# Autodesk Inventor assembly: inner
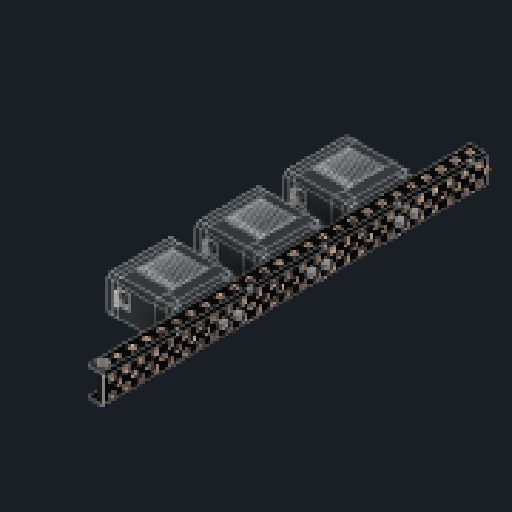
[picture p0: Inventor's stored thumbnail of the model, 512x512]
Saved by Autodesk Inventor 2024 (Build 280153000, 153)
## iProperties
Created: 2024-03-23
Part Number: inner
Document SubType Name: Assembly
Designer: Averey Ku
Author: Averey Ku
## Documents named in this file (8)
- D:\vex_robotics\hardware\cad\infection\chassis\drivebay\inner.iam
- D:\vex_robotics\hardware\cad\VEX-CAD-Inventor-1.41\Structure\Standoff\Standoff .875.ipt
- D:\vex_robotics\hardware\cad\VEX-CAD-Inventor-1.41\Structure\Standoff.ipt
- D:\vex_robotics\hardware\cad\VEX-CAD-Inventor-1.41\Motion\Spacers\Washer Steel\SWasher .375 OD x .062500.ipt
- D:\vex_robotics\hardware\cad\VEX-CAD-Inventor-1.41\Motion\Spacers\Washer Steel.ipt
- D:\vex_robotics\hardware\cad\VEX-CAD-Inventor-1.41\Electronics\V5 Motor.ipt
- D:\vex_robotics\hardware\cad\hardware\Nylon Screw Pan-Head .500.ipt
- D:\vex_robotics\hardware\cad\VEX-CAD-Inventor-1.41\Structure\C Channel\Aluminum 1x2x1\Alu C 1x2x1x26.ipt
## Components (12 placed, 5 different names)
1. Standoff .875:1 — Insert:10
2. SWasher .375 OD x .062500:1 — Insert:9
3. V5 Motor:1 — Insert:3, Insert:4
4. Nylon Screw Pan-Head .500:1 — Insert:4, Mate:3
5. Nylon Screw Pan-Head .500:2 — Insert:3, Insert:13
6. V5 Motor:2
7. Nylon Screw Pan-Head .500:3 — Insert:11
8. Nylon Screw Pan-Head .500:4 — Mate:1
9. V5 Motor:3
10. Nylon Screw Pan-Head .500:5 — Insert:12
11. Nylon Screw Pan-Head .500:6 — Mate:2
12. Alu C 1x2x1x26:1 — Insert:9, Insert:10, Insert:11, Mate:1, Insert:12, Mate:2, Insert:13, Mate:3
## Relationships (14: Insert 11, Mate 3)
- Insert:3 (1.5875 mm): V5 Motor:1 ↔ Nylon Screw Pan-Head .500:2
- Insert:4 (1.5875 mm): V5 Motor:1 ↔ Nylon Screw Pan-Head .500:1
- [Insert] (1.5875 mm): V5 Motor:2 ↔ Nylon Screw Pan-Head .500:4
- [Insert] (1.5875 mm): V5 Motor:2 ↔ Nylon Screw Pan-Head .500:3
- [Insert] (1.5875 mm): V5 Motor:3 ↔ Nylon Screw Pan-Head .500:6
- [Insert] (1.5875 mm): V5 Motor:3 ↔ Nylon Screw Pan-Head .500:5
- Insert:9: SWasher .375 OD x .062500:1 ↔ Alu C 1x2x1x26:1
- Insert:10: Standoff .875:1 ↔ Alu C 1x2x1x26:1
- Insert:11: Nylon Screw Pan-Head .500:3 ↔ Alu C 1x2x1x26:1
- Mate:1: Nylon Screw Pan-Head .500:4 ↔ Alu C 1x2x1x26:1
- Insert:12: Nylon Screw Pan-Head .500:5 ↔ Alu C 1x2x1x26:1
- Mate:2: Nylon Screw Pan-Head .500:6 ↔ Alu C 1x2x1x26:1
- Insert:13: Nylon Screw Pan-Head .500:2 ↔ Alu C 1x2x1x26:1
- Mate:3: Nylon Screw Pan-Head .500:1 ↔ Alu C 1x2x1x26:1
## Named parameters: d4_d2 = 1.5875 mm, d5_d3 = 1.5875 mm, d6_d2 = 1.5875 mm, d7_d3 = 1.5875 mm
